# Autodesk Inventor assembly: motor_25kg
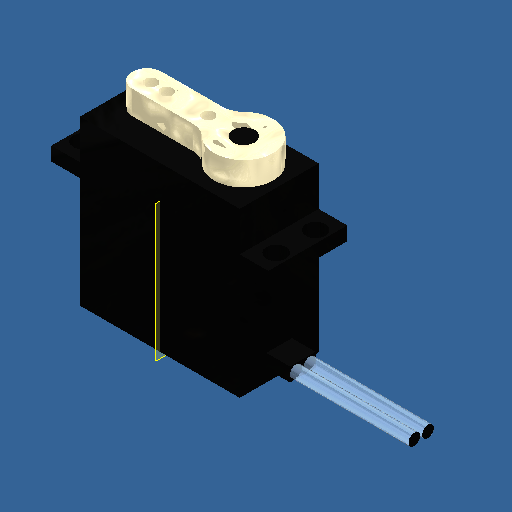
[picture p0: Inventor's stored thumbnail of the model, 512x512]
Saved by Autodesk Inventor 2025 (Build 290162000, 162)
## iProperties
Created: 2024-12-10
Part Number: motor_25kg
Document SubType Name: Assembly
Designer: Pauline Simonnet
Author: Pauline Simonnet
## Documents named in this file (3)
- C:\Users\Pauline Simonnet\Documents\ISAE SUPAERO\SupaeroMoon\MDRS\components\motor_25kg.iam
- C:\Users\Pauline Simonnet\Documents\ISAE SUPAERO\SupaeroMoon\MDRS\components\motor_25kg.ipt
- C:\Users\Pauline Simonnet\Documents\ISAE SUPAERO\SupaeroMoon\MDRS\components\adaptator_25.ipt
## Components (2 placed, 2 different names)
1. motor_25kg:1 — Mate:1, Flush:1
2. adaptator_25:1 — Mate:1, Flush:1
## Relationships (2: Mate 1, Flush 1)
- Mate:1: motor_25kg:1 ↔ adaptator_25:1
- Flush:1: motor_25kg:1 ↔ adaptator_25:1
